# Autodesk Inventor assembly: Backpack
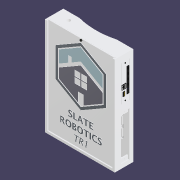
[picture p0: Inventor's stored thumbnail of the model, 180x180]
Saved by Autodesk Inventor 2017 SP1 (Build 210196100, 196)
## iProperties
Created: 2017-09-05
Part Number: Backpack
Document SubType Name: Assembly
Designer: Zach
Author: Zach
## Documents named in this file (18)
- C:\Users\Zach\Documents\GitHub\tr1\src\Body\Chest Assembly\Backpack Assembly\Backpack.iam
- C:\Users\Zach\Documents\GitHub\tr1\src\Body\Chest Assembly\Backpack Assembly\BP001b.ipt
- C:\Users\Zach\Documents\GitHub\tr1\src\Body\Chest Assembly\Backpack Assembly\BP002b.ipt
- C:\Users\Zach\Documents\GitHub\tr1\src\Body\Chest Assembly\Backpack Assembly\BP003.ipt
- C:\Users\Zach\Documents\GitHub\tr1\src\Body\Chest Assembly\Backpack Assembly\BP005.ipt
- C:\Users\Zach\Documents\GitHub\tr1\src\Body\Chest Assembly\Backpack Assembly\BP006.ipt
- C:\Users\Zach\Documents\GitHub\tr1\lib\Terminal Block 4\Клемная колодка ТВ-2504L 600V-25A\Клемная колодка ТВ-2504L 600V-25A.iam
- C:\Users\Zach\Documents\GitHub\tr1\lib\Arduino Mega 2560\Arduino Mega 2560.ipt
- C:\Users\Zach\Documents\GitHub\tr1\lib\L298n H Bridge\L298N\07j5423_1546306-8.ipt
- C:\Users\Zach\Documents\GitHub\tr1\lib\L298n Driver\l298n.ipt
- C:\Users\Zach\Documents\Inventor\Content Center Files\R2017\en-US\ISO 7045  H\ISO 7045 - M3 x 12 - 4.8 - H - ISO.ipt
- C:\Users\Zach\Documents\Inventor\Content Center Files\R2017\en-US\ISO 4018\ISO 4018 - M5 x 25.ipt
- C:\Users\Zach\Documents\GitHub\tr1\src\Body\Chest Assembly\Backpack Assembly\BP010.ipt
- C:\Users\Zach\Documents\GitHub\tr1\src\Body\Chest Assembly\Backpack Assembly\USB Hub.ipt
- C:\Users\Zach\Documents\GitHub\tr1\src\Body\Chest Assembly\Backpack Assembly\HDMI Port.ipt
- C:\Users\Zach\Documents\GitHub\tr1\src\Body\Chest Assembly\Backpack Assembly\Ethernet Port.ipt
- C:\Users\Zach\Documents\GitHub\tr1\src\Body\Chest Assembly\Backpack Assembly\SD Port.ipt
- C:\Users\Zach\Documents\Inventor\Content Center Files\R2017\en-US\ISO 4035(2)\ISO 4035 - M3 - ISO.ipt
## Components (92 placed, 17 different names)
1. BP001b:1 — Mate:8, Mate:9, Mate:11, Mate:13, Mate:15, Mate:19, Mate:20, Mate:21, Mate:22, Mate:23, Flush:1, Mate:24, Mate:25, Mate:26, Mate:36, Mate:37, Mate:38, Mate:39, Mate:56, Mate:57, Mate:58, Mate:133, Mate:134, Mate:137, Mate:138, Mate:141, Mate:142, Mate:145, Mate:146, Mate:149, Mate:150, Mate:160, Mate:162, Mate:163, Mate:176, Mate:177, Mate:178, Mate:179, Mate:180, Mate:181, Mate:182, Mate:183, Mate:184, Mate:185, Mate:186, Mate:187, Mate:188, Mate:189, Mate:190, Mate:191, Mate:270, Mate:271, Mate:272, Mate:280, Mate:310, Mate:312, Mate:314, Mate:316, Mate:317, Mate:318, Mate:319, Mate:326, Mate:327, Mate:328, Mate:330, Mate:331, Mate:332
2. BP002b:1 — Mate:317, Mate:318, Mate:319, Mate:333
3. BP003:1 — Mate:15, Mate:36, Mate:37, Mate:65, Mate:66, Mate:67, Mate:68, Mate:69, Mate:70, Mate:135, Mate:136, Mate:232, Mate:233, Mate:234, Mate:235, Mate:236, Mate:237, Mate:238, Mate:239, Mate:240, Mate:241, Mate:242, Mate:243
4. BP003:2 — Mate:19, Mate:38, Mate:39, Mate:59, Mate:60, Mate:61, Mate:62, Mate:63, Mate:64, Mate:139, Mate:140, Mate:208, Mate:209, Mate:210, Mate:211, Mate:212, Mate:213, Mate:214, Mate:215, Mate:216, Mate:217, Mate:218, Mate:219
5. BP005:1 — Mate:8, Mate:9, Mate:20, Mate:172, Mate:173, Mate:174, Mate:175, Flush:9, Mate:287, Mate:288, Mate:307, Mate:308
6. BP006:1 — Mate:11, Mate:13, Mate:21, Mate:168, Mate:169, Mate:170, Mate:171, Flush:6, Mate:282, Mate:283, Flush:7, Mate:284, Mate:285, Flush:8, Mate:286
7. BP010:1 — Mate:270, Mate:271, Mate:272, Mate:273, Mate:274, Mate:275, Mate:276, Mate:277, Mate:278, Mate:279
8. Клемная колодка ТВ-2504L 600V-25A:1 [sub-assembly] — Mate:24, Mate:25, Mate:26, Mate:151, Mate:152
9. Arduino Mega 2560:1 — Mate:96, Mate:116, Mate:117, Mate:118, Mate:119, Mate:120, Mate:327, Mate:328, Mate:329
10. Arduino Mega 2560:2 — Mate:127, Mate:128, Mate:129, Mate:130, Mate:131, Mate:132, Mate:326, Mate:330, Mate:331
11. 07j5423_1546306-8:1 — Mate:56, Mate:57, Mate:58, Mate:143, Mate:144, Mate:147, Mate:148
12. l298n:1 — Mate:59, Mate:60, Flush:3, Mate:228, Mate:229, Mate:230, Mate:231
13. l298n:2 — Mate:62, Mate:63, Flush:2, Flush:3, Mate:224, Mate:225, Mate:226, Mate:227
14. l298n:3 — Mate:61, Mate:64, Flush:2, Mate:220, Mate:221, Mate:222, Mate:223
15. l298n:4 — Mate:67, Mate:70, Flush:4, Flush:5, Mate:248, Mate:249, Mate:250, Mate:251
16. l298n:5 — Mate:68, Mate:69, Flush:5, Mate:252, Mate:253, Mate:254, Mate:255
17. l298n:6 — Mate:65, Mate:66, Flush:4, Mate:244, Mate:245, Mate:246, Mate:247
18. USB Hub:1 — Mate:280, Flush:6, Mate:286
19. HDMI Port:1 — Mate:282, Mate:283, Flush:7
20. Ethernet Port:1 — Mate:284, Mate:285, Flush:8
21. SD Port:1 — Flush:9, Mate:287, Mate:288
22. ISO 7045 H M3 x 12 - 4.8 - H:1 — Mate:96, Mate:329
23. ISO 7045 H M3 x 12 - 4.8 - H:2 — Mate:117
24. ISO 7045 H M3 x 12 - 4.8 - H:3 — Mate:119
25. ISO 7045 H M3 x 12 - 4.8 - H:4 — Mate:120
26. ISO 7045 H M3 x 12 - 4.8 - H:5 — Mate:118
27. ISO 7045 H M3 x 12 - 4.8 - H:6 — Mate:116
28. ISO 7045 H M3 x 12 - 4.8 - H:7 — Mate:128
29. ISO 7045 H M3 x 12 - 4.8 - H:8 — Mate:131
30. ISO 7045 H M3 x 12 - 4.8 - H:9 — Mate:132
31. ISO 7045 H M3 x 12 - 4.8 - H:10 — Mate:129
32. ISO 7045 H M3 x 12 - 4.8 - H:11 — Mate:130
33. ISO 7045 H M3 x 12 - 4.8 - H:12 — Mate:127
34. ISO 7045 H M3 x 12 - 4.8 - H:13 — Mate:133, Mate:136
35. ISO 7045 H M3 x 12 - 4.8 - H:14 — Mate:134, Mate:135
36. ISO 7045 H M3 x 12 - 4.8 - H:15 — Mate:137, Mate:139
37. ISO 7045 H M3 x 12 - 4.8 - H:16 — Mate:138, Mate:140
38. ISO 7045 H M3 x 12 - 4.8 - H:17 — Mate:142, Mate:143
39. ISO 7045 H M3 x 12 - 4.8 - H:18 — Mate:141, Mate:144
40. ISO 7045 H M3 x 12 - 4.8 - H:19 — Mate:146, Mate:148
41. ISO 7045 H M3 x 12 - 4.8 - H:20 — Mate:145, Mate:147
42. ISO 7045 H M3 x 12 - 4.8 - H:21 — Mate:149, Mate:152
43. ISO 7045 H M3 x 12 - 4.8 - H:22 — Mate:150, Mate:151
44. ISO 7045 H M3 x 12 - 4.8 - H:27 — Mate:160
45. ISO 7045 H M3 x 12 - 4.8 - H:28 — Mate:163
46. ISO 7045 H M3 x 12 - 4.8 - H:30 — Mate:162
47. ISO 7045 H M3 x 12 - 4.8 - H:31 — Mate:169, Mate:170, Mate:313
48. ISO 7045 H M3 x 12 - 4.8 - H:32 — Mate:168, Mate:171, Mate:315
49. ISO 7045 H M3 x 12 - 4.8 - H:33 — Mate:172, Mate:173, Mate:309
50. ISO 7045 H M3 x 12 - 4.8 - H:34 — Mate:174, Mate:175
51. ISO 4018 M5 x 25:5 — Mate:179, Mate:190
52. ISO 4018 M5 x 25:6 — Mate:181, Mate:186
53. ISO 4018 M5 x 25:7 — Mate:182, Mate:187
54. ISO 4018 M5 x 25:8 — Mate:180, Mate:189
55. ISO 4018 M5 x 25:9 — Mate:177, Mate:191
56. ISO 4018 M5 x 25:10 — Mate:176, Mate:184
57. ISO 4018 M5 x 25:11 — Mate:178, Mate:185
58. ISO 4018 M5 x 25:12 — Mate:183, Mate:188
59. ISO 7045 H M3 x 12 - 4.8 - H:35 — Mate:219, Mate:230
60. ISO 7045 H M3 x 12 - 4.8 - H:36 — Mate:218, Mate:229
61. ISO 7045 H M3 x 12 - 4.8 - H:37 — Mate:217, Mate:228
62. ISO 7045 H M3 x 12 - 4.8 - H:38 — Mate:215, Mate:225
63. ISO 7045 H M3 x 12 - 4.8 - H:39 — Mate:216, Mate:231
64. ISO 7045 H M3 x 12 - 4.8 - H:40 — Mate:214, Mate:224
65. ISO 7045 H M3 x 12 - 4.8 - H:41 — Mate:213, Mate:226
66. ISO 7045 H M3 x 12 - 4.8 - H:42 — Mate:211, Mate:222
67. ISO 7045 H M3 x 12 - 4.8 - H:43 — Mate:210, Mate:223
68. ISO 7045 H M3 x 12 - 4.8 - H:44 — Mate:212, Mate:227
69. ISO 7045 H M3 x 12 - 4.8 - H:45 — Mate:209, Mate:220
70. ISO 7045 H M3 x 12 - 4.8 - H:46 — Mate:208, Mate:221
71. ISO 7045 H M3 x 12 - 4.8 - H:47 — Mate:238, Mate:248
72. ISO 7045 H M3 x 12 - 4.8 - H:48 — Mate:239, Mate:250
73. ISO 7045 H M3 x 12 - 4.8 - H:49 — Mate:243, Mate:254
74. ISO 7045 H M3 x 12 - 4.8 - H:50 — Mate:242, Mate:255
75. ISO 7045 H M3 x 12 - 4.8 - H:51 — Mate:232, Mate:245
76. ISO 7045 H M3 x 12 - 4.8 - H:52 — Mate:233, Mate:244
77. ISO 7045 H M3 x 12 - 4.8 - H:53 — Mate:235, Mate:246
78. ISO 7045 H M3 x 12 - 4.8 - H:54 — Mate:234, Mate:247
79. ISO 7045 H M3 x 12 - 4.8 - H:55 — Mate:236, Mate:249
80. ISO 7045 H M3 x 12 - 4.8 - H:56 — Mate:237, Mate:251
81. ISO 7045 H M3 x 12 - 4.8 - H:57 — Mate:240, Mate:253
82. ISO 7045 H M3 x 12 - 4.8 - H:58 — Mate:241, Mate:252
83. ISO 7045 H M3 x 12 - 4.8 - H:63 — Mate:273
84. ISO 7045 H M3 x 12 - 4.8 - H:64 — Mate:274, Mate:277
85. ISO 7045 H M3 x 12 - 4.8 - H:65 — Mate:275, Mate:278
86. ISO 7045 H M3 x 12 - 4.8 - H:66 — Mate:276, Mate:279
87. ISO 7045 H M3 x 12 - 4.8 - H:67 — Mate:307, Mate:308, Mate:311
88. ISO 4035 M3:1 — Mate:309, Mate:310
89. ISO 4035 M3:2 — Mate:311, Mate:312
90. ISO 4035 M3:3 — Mate:313, Mate:314
91. ISO 4035 M3:4 — Mate:315, Mate:316
92. ISO 4018 M5 x 25:13 — Mate:332, Mate:333
## Relationships (187: Mate 178, Flush 9)
- Mate:8: BP001b:1 ↔ BP005:1
- Mate:9: BP001b:1 ↔ BP005:1
- Mate:11: BP001b:1 ↔ BP006:1
- Mate:13: BP001b:1 ↔ BP006:1
- Mate:15: BP001b:1 ↔ BP003:1
- Mate:19: BP001b:1 ↔ BP003:2
- Mate:20: BP001b:1 ↔ BP005:1
- Mate:21: BP001b:1 ↔ BP006:1
- Mate:22: BP001b:1
- Mate:23: BP001b:1
- Flush:1 (200 mm): BP001b:1
- Mate:24: BP001b:1 ↔ Клемная колодка ТВ-2504L 600V-25A:1
- Mate:25: BP001b:1 ↔ Клемная колодка ТВ-2504L 600V-25A:1
- Mate:26: BP001b:1 ↔ Клемная колодка ТВ-2504L 600V-25A:1
- Mate:36: BP001b:1 ↔ BP003:1
- Mate:37: BP001b:1 ↔ BP003:1
- Mate:38: BP001b:1 ↔ BP003:2
- Mate:39: BP001b:1 ↔ BP003:2
- Mate:56: BP001b:1 ↔ 07j5423_1546306-8:1
- Mate:57: BP001b:1 ↔ 07j5423_1546306-8:1
- Mate:58: BP001b:1 ↔ 07j5423_1546306-8:1
- Mate:59: BP003:2 ↔ l298n:1
- Mate:60: BP003:2 ↔ l298n:1
- Mate:61: BP003:2 ↔ l298n:3
- Mate:62: BP003:2 ↔ l298n:2
- Mate:63: BP003:2 ↔ l298n:2
- Mate:64: BP003:2 ↔ l298n:3
- Flush:2: l298n:2 ↔ l298n:3
- Flush:3: l298n:1 ↔ l298n:2
- Mate:65: BP003:1 ↔ l298n:6
- Mate:66: BP003:1 ↔ l298n:6
- Mate:67: BP003:1 ↔ l298n:4
- Mate:68: BP003:1 ↔ l298n:5
- Mate:69: BP003:1 ↔ l298n:5
- Mate:70: BP003:1 ↔ l298n:4
- Flush:4: l298n:4 ↔ l298n:6
- Flush:5: l298n:4 ↔ l298n:5
- Mate:96: Arduino Mega 2560:1 ↔ ISO 7045 H M3 x 12 - 4.8 - H:1
- Mate:116: Arduino Mega 2560:1 ↔ ISO 7045 H M3 x 12 - 4.8 - H:6
- Mate:117: Arduino Mega 2560:1 ↔ ISO 7045 H M3 x 12 - 4.8 - H:2
- Mate:118: Arduino Mega 2560:1 ↔ ISO 7045 H M3 x 12 - 4.8 - H:5
- Mate:119: Arduino Mega 2560:1 ↔ ISO 7045 H M3 x 12 - 4.8 - H:3
- Mate:120: Arduino Mega 2560:1 ↔ ISO 7045 H M3 x 12 - 4.8 - H:4
- Mate:127: Arduino Mega 2560:2 ↔ ISO 7045 H M3 x 12 - 4.8 - H:12
- Mate:128: Arduino Mega 2560:2 ↔ ISO 7045 H M3 x 12 - 4.8 - H:7
- Mate:129: Arduino Mega 2560:2 ↔ ISO 7045 H M3 x 12 - 4.8 - H:10
- Mate:130: Arduino Mega 2560:2 ↔ ISO 7045 H M3 x 12 - 4.8 - H:11
- Mate:131: Arduino Mega 2560:2 ↔ ISO 7045 H M3 x 12 - 4.8 - H:8
- Mate:132: Arduino Mega 2560:2 ↔ ISO 7045 H M3 x 12 - 4.8 - H:9
- Mate:133: BP001b:1 ↔ ISO 7045 H M3 x 12 - 4.8 - H:13
- Mate:134: BP001b:1 ↔ ISO 7045 H M3 x 12 - 4.8 - H:14
- Mate:135: BP003:1 ↔ ISO 7045 H M3 x 12 - 4.8 - H:14
- Mate:136: BP003:1 ↔ ISO 7045 H M3 x 12 - 4.8 - H:13
- Mate:137: BP001b:1 ↔ ISO 7045 H M3 x 12 - 4.8 - H:15
- Mate:138: BP001b:1 ↔ ISO 7045 H M3 x 12 - 4.8 - H:16
- Mate:139: BP003:2 ↔ ISO 7045 H M3 x 12 - 4.8 - H:15
- Mate:140: BP003:2 ↔ ISO 7045 H M3 x 12 - 4.8 - H:16
- Mate:141: BP001b:1 ↔ ISO 7045 H M3 x 12 - 4.8 - H:18
- Mate:142: BP001b:1 ↔ ISO 7045 H M3 x 12 - 4.8 - H:17
- Mate:143: 07j5423_1546306-8:1 ↔ ISO 7045 H M3 x 12 - 4.8 - H:17
- Mate:144: 07j5423_1546306-8:1 ↔ ISO 7045 H M3 x 12 - 4.8 - H:18
- Mate:145: BP001b:1 ↔ ISO 7045 H M3 x 12 - 4.8 - H:20
- Mate:146: BP001b:1 ↔ ISO 7045 H M3 x 12 - 4.8 - H:19
- Mate:147: 07j5423_1546306-8:1 ↔ ISO 7045 H M3 x 12 - 4.8 - H:20
- Mate:148: 07j5423_1546306-8:1 ↔ ISO 7045 H M3 x 12 - 4.8 - H:19
- Mate:149: BP001b:1 ↔ ISO 7045 H M3 x 12 - 4.8 - H:21
- Mate:150: BP001b:1 ↔ ISO 7045 H M3 x 12 - 4.8 - H:22
- Mate:151: Клемная колодка ТВ-2504L 600V-25A:1 ↔ ISO 7045 H M3 x 12 - 4.8 - H:22
- Mate:152: Клемная колодка ТВ-2504L 600V-25A:1 ↔ ISO 7045 H M3 x 12 - 4.8 - H:21
- Mate:160: BP001b:1 ↔ ISO 7045 H M3 x 12 - 4.8 - H:27
- Mate:162: BP001b:1 ↔ ISO 7045 H M3 x 12 - 4.8 - H:30
- Mate:163: BP001b:1 ↔ ISO 7045 H M3 x 12 - 4.8 - H:28
- Mate:168: BP006:1 ↔ ISO 7045 H M3 x 12 - 4.8 - H:32
- Mate:169: BP006:1 ↔ ISO 7045 H M3 x 12 - 4.8 - H:31
- Mate:170: BP006:1 ↔ ISO 7045 H M3 x 12 - 4.8 - H:31
- Mate:171: BP006:1 ↔ ISO 7045 H M3 x 12 - 4.8 - H:32
- Mate:172: BP005:1 ↔ ISO 7045 H M3 x 12 - 4.8 - H:33
- Mate:173: BP005:1 ↔ ISO 7045 H M3 x 12 - 4.8 - H:33
- Mate:174: BP005:1 ↔ ISO 7045 H M3 x 12 - 4.8 - H:34
- Mate:175: BP005:1 ↔ ISO 7045 H M3 x 12 - 4.8 - H:34
- Mate:176: BP001b:1 ↔ ISO 4018 M5 x 25:10
- Mate:177: BP001b:1 ↔ ISO 4018 M5 x 25:9
- Mate:178: BP001b:1 ↔ ISO 4018 M5 x 25:11
- Mate:179: BP001b:1 ↔ ISO 4018 M5 x 25:5
- Mate:180: BP001b:1 ↔ ISO 4018 M5 x 25:8
- Mate:181: BP001b:1 ↔ ISO 4018 M5 x 25:6
- Mate:182: BP001b:1 ↔ ISO 4018 M5 x 25:7
- Mate:183: BP001b:1 ↔ ISO 4018 M5 x 25:12
- Mate:184: BP001b:1 ↔ ISO 4018 M5 x 25:10
- Mate:185: BP001b:1 ↔ ISO 4018 M5 x 25:11
- Mate:186: BP001b:1 ↔ ISO 4018 M5 x 25:6
- Mate:187: BP001b:1 ↔ ISO 4018 M5 x 25:7
- Mate:188: BP001b:1 ↔ ISO 4018 M5 x 25:12
- Mate:189: BP001b:1 ↔ ISO 4018 M5 x 25:8
- Mate:190: BP001b:1 ↔ ISO 4018 M5 x 25:5
- Mate:191: BP001b:1 ↔ ISO 4018 M5 x 25:9
- Mate:208: BP003:2 ↔ ISO 7045 H M3 x 12 - 4.8 - H:46
- Mate:209: BP003:2 ↔ ISO 7045 H M3 x 12 - 4.8 - H:45
- Mate:210: BP003:2 ↔ ISO 7045 H M3 x 12 - 4.8 - H:43
- Mate:211: BP003:2 ↔ ISO 7045 H M3 x 12 - 4.8 - H:42
- Mate:212: BP003:2 ↔ ISO 7045 H M3 x 12 - 4.8 - H:44
- Mate:213: BP003:2 ↔ ISO 7045 H M3 x 12 - 4.8 - H:41
- Mate:214: BP003:2 ↔ ISO 7045 H M3 x 12 - 4.8 - H:40
- Mate:215: BP003:2 ↔ ISO 7045 H M3 x 12 - 4.8 - H:38
- Mate:216: BP003:2 ↔ ISO 7045 H M3 x 12 - 4.8 - H:39
- Mate:217: BP003:2 ↔ ISO 7045 H M3 x 12 - 4.8 - H:37
- Mate:218: BP003:2 ↔ ISO 7045 H M3 x 12 - 4.8 - H:36
- Mate:219: BP003:2 ↔ ISO 7045 H M3 x 12 - 4.8 - H:35
- Mate:220: l298n:3 ↔ ISO 7045 H M3 x 12 - 4.8 - H:45
- Mate:221: l298n:3 ↔ ISO 7045 H M3 x 12 - 4.8 - H:46
- Mate:222: l298n:3 ↔ ISO 7045 H M3 x 12 - 4.8 - H:42
- Mate:223: l298n:3 ↔ ISO 7045 H M3 x 12 - 4.8 - H:43
- Mate:224: l298n:2 ↔ ISO 7045 H M3 x 12 - 4.8 - H:40
- Mate:225: l298n:2 ↔ ISO 7045 H M3 x 12 - 4.8 - H:38
- Mate:226: l298n:2 ↔ ISO 7045 H M3 x 12 - 4.8 - H:41
- Mate:227: l298n:2 ↔ ISO 7045 H M3 x 12 - 4.8 - H:44
- Mate:228: l298n:1 ↔ ISO 7045 H M3 x 12 - 4.8 - H:37
- Mate:229: l298n:1 ↔ ISO 7045 H M3 x 12 - 4.8 - H:36
- Mate:230: l298n:1 ↔ ISO 7045 H M3 x 12 - 4.8 - H:35
- Mate:231: l298n:1 ↔ ISO 7045 H M3 x 12 - 4.8 - H:39
- Mate:232: BP003:1 ↔ ISO 7045 H M3 x 12 - 4.8 - H:51
- Mate:233: BP003:1 ↔ ISO 7045 H M3 x 12 - 4.8 - H:52
- Mate:234: BP003:1 ↔ ISO 7045 H M3 x 12 - 4.8 - H:54
- Mate:235: BP003:1 ↔ ISO 7045 H M3 x 12 - 4.8 - H:53
- Mate:236: BP003:1 ↔ ISO 7045 H M3 x 12 - 4.8 - H:55
- Mate:237: BP003:1 ↔ ISO 7045 H M3 x 12 - 4.8 - H:56
- Mate:238: BP003:1 ↔ ISO 7045 H M3 x 12 - 4.8 - H:47
- Mate:239: BP003:1 ↔ ISO 7045 H M3 x 12 - 4.8 - H:48
- Mate:240: BP003:1 ↔ ISO 7045 H M3 x 12 - 4.8 - H:57
- Mate:241: BP003:1 ↔ ISO 7045 H M3 x 12 - 4.8 - H:58
- Mate:242: BP003:1 ↔ ISO 7045 H M3 x 12 - 4.8 - H:50
- Mate:243: BP003:1 ↔ ISO 7045 H M3 x 12 - 4.8 - H:49
- Mate:244: l298n:6 ↔ ISO 7045 H M3 x 12 - 4.8 - H:52
- Mate:245: l298n:6 ↔ ISO 7045 H M3 x 12 - 4.8 - H:51
- Mate:246: l298n:6 ↔ ISO 7045 H M3 x 12 - 4.8 - H:53
- Mate:247: l298n:6 ↔ ISO 7045 H M3 x 12 - 4.8 - H:54
- Mate:248: l298n:4 ↔ ISO 7045 H M3 x 12 - 4.8 - H:47
- Mate:249: l298n:4 ↔ ISO 7045 H M3 x 12 - 4.8 - H:55
- Mate:250: l298n:4 ↔ ISO 7045 H M3 x 12 - 4.8 - H:48
- Mate:251: l298n:4 ↔ ISO 7045 H M3 x 12 - 4.8 - H:56
- Mate:252: l298n:5 ↔ ISO 7045 H M3 x 12 - 4.8 - H:58
- Mate:253: l298n:5 ↔ ISO 7045 H M3 x 12 - 4.8 - H:57
- Mate:254: l298n:5 ↔ ISO 7045 H M3 x 12 - 4.8 - H:49
- Mate:255: l298n:5 ↔ ISO 7045 H M3 x 12 - 4.8 - H:50
- Mate:270: BP001b:1 ↔ BP010:1
- Mate:271: BP001b:1 ↔ BP010:1
- Mate:272: BP001b:1 ↔ BP010:1
- Mate:273: BP010:1 ↔ ISO 7045 H M3 x 12 - 4.8 - H:63
- Mate:274: BP010:1 ↔ ISO 7045 H M3 x 12 - 4.8 - H:64
- Mate:275: BP010:1 ↔ ISO 7045 H M3 x 12 - 4.8 - H:65
- Mate:276: BP010:1 ↔ ISO 7045 H M3 x 12 - 4.8 - H:66
- Mate:277: BP010:1 ↔ ISO 7045 H M3 x 12 - 4.8 - H:64
- Mate:278: BP010:1 ↔ ISO 7045 H M3 x 12 - 4.8 - H:65
- Mate:279: BP010:1 ↔ ISO 7045 H M3 x 12 - 4.8 - H:66
- Mate:280: BP001b:1 ↔ USB Hub:1
- Flush:6: BP006:1 ↔ USB Hub:1
- Mate:282 (0.5 mm): BP006:1 ↔ HDMI Port:1
- Mate:283 (0.5 mm): BP006:1 ↔ HDMI Port:1
- Flush:7: BP006:1 ↔ HDMI Port:1
- Mate:284: BP006:1 ↔ Ethernet Port:1
- Mate:285 (0.5 mm): BP006:1 ↔ Ethernet Port:1
- Flush:8: BP006:1 ↔ Ethernet Port:1
- Mate:286 (0.5 mm): BP006:1 ↔ USB Hub:1
- Flush:9: BP005:1 ↔ SD Port:1
- Mate:287 (0.5 mm): BP005:1 ↔ SD Port:1
- Mate:288 (0.5 mm): BP005:1 ↔ SD Port:1
- Mate:307: BP005:1 ↔ ISO 7045 H M3 x 12 - 4.8 - H:67
- Mate:308: BP005:1 ↔ ISO 7045 H M3 x 12 - 4.8 - H:67
- Mate:309: ISO 7045 H M3 x 12 - 4.8 - H:33 ↔ ISO 4035 M3:1
- Mate:310: BP001b:1 ↔ ISO 4035 M3:1
- Mate:311: ISO 7045 H M3 x 12 - 4.8 - H:67 ↔ ISO 4035 M3:2
- Mate:312: BP001b:1 ↔ ISO 4035 M3:2
- Mate:313: ISO 7045 H M3 x 12 - 4.8 - H:31 ↔ ISO 4035 M3:3
- Mate:314: BP001b:1 ↔ ISO 4035 M3:3
- Mate:315: ISO 7045 H M3 x 12 - 4.8 - H:32 ↔ ISO 4035 M3:4
- Mate:316: BP001b:1 ↔ ISO 4035 M3:4
- Mate:317: BP001b:1 ↔ BP002b:1
- Mate:318 (1 mm): BP001b:1 ↔ BP002b:1
- Mate:319: BP001b:1 ↔ BP002b:1
- Mate:326: BP001b:1 ↔ Arduino Mega 2560:2
- Mate:327: BP001b:1 ↔ Arduino Mega 2560:1
- Mate:328: BP001b:1 ↔ Arduino Mega 2560:1
- Mate:329: Arduino Mega 2560:1 ↔ ISO 7045 H M3 x 12 - 4.8 - H:1
- Mate:330: BP001b:1 ↔ Arduino Mega 2560:2
- Mate:331: BP001b:1 ↔ Arduino Mega 2560:2
- Mate:332: BP001b:1 ↔ ISO 4018 M5 x 25:13
- Mate:333: BP002b:1 ↔ ISO 4018 M5 x 25:13
